# Autodesk Inventor assembly: ODSY-0003-100
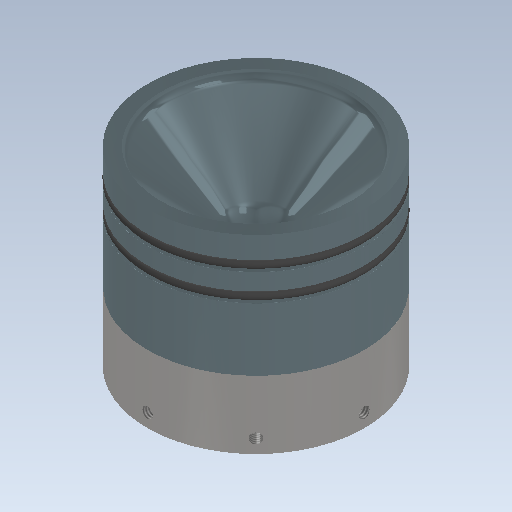
[picture p0: Inventor's stored thumbnail of the model, 512x512]
Saved by Autodesk Inventor 2021 (Build 250183000, 183)
## iProperties
Company: ERPL
Created: 2021-10-19
Document SubType Name: Assembly
Designer: ALEX CLAY
Project: ODYSSEY
Description: NOZZLE ASSEMBLY
Mass: 1940.44 g
Surface Area: 815.338 cm^2
Volume: 571.29 cm^3
Density: 3.39659 g/cm^3
Author: ALEX CLAY
Revision Number: 00
## Documents named in this file (4)
- C:\Users\alexc\OneDrive\Desktop\ATLAS\ODSY-0003 (COMBUSTION CHAMBER)\ODSY-0003-100 (NOZZLE)\ODSY-0003-100.iam
- C:\Users\alexc\OneDrive\Desktop\ATLAS\ODSY-0003 (COMBUSTION CHAMBER)\ODSY-0003-100 (NOZZLE)\ODSY-0003-101.ipt
- C:\Users\alexc\OneDrive\Desktop\ATLAS\ODSY-0003 (COMBUSTION CHAMBER)\ODSY-0003-100 (NOZZLE)\ODSY-0003-102.ipt
- C:\Users\alexc\OneDrive\Desktop\ATLAS\ODSY-0003 (COMBUSTION CHAMBER)\ODSY-0003-100 (NOZZLE)\2-240.ipt
## Components (4 placed, 3 different names)
1. ODSY-0003-101:1 — Mate:1, Mate:2, Mate:3, Mate:4, Flush:1, Mate:5
2. ODSY-0003-102:1 — Mate:4, Flush:1, Mate:5, Mate:6, Mate:7, Flush:2, Mate:8
3. 2-240:1 — Mate:6, Flush:2, Mate:9
4. 2-240:2 — Mate:7, Mate:8, Flush:3
## Relationships (12: Mate 9, Flush 3)
- Mate:1: ODSY-0003-101:1
- Mate:2: ODSY-0003-101:1
- Mate:3: ODSY-0003-101:1
- Mate:4: ODSY-0003-101:1 ↔ ODSY-0003-102:1
- Flush:1: ODSY-0003-101:1 ↔ ODSY-0003-102:1
- Mate:5: ODSY-0003-101:1 ↔ ODSY-0003-102:1
- Mate:6: ODSY-0003-102:1 ↔ 2-240:1
- Mate:7: ODSY-0003-102:1 ↔ 2-240:2
- Flush:2: ODSY-0003-102:1 ↔ 2-240:1
- Mate:8: ODSY-0003-102:1 ↔ 2-240:2
- Mate:9: 2-240:1
- Flush:3: 2-240:2
